# Autodesk Inventor assembly: ASY MSC 900.6 base frame
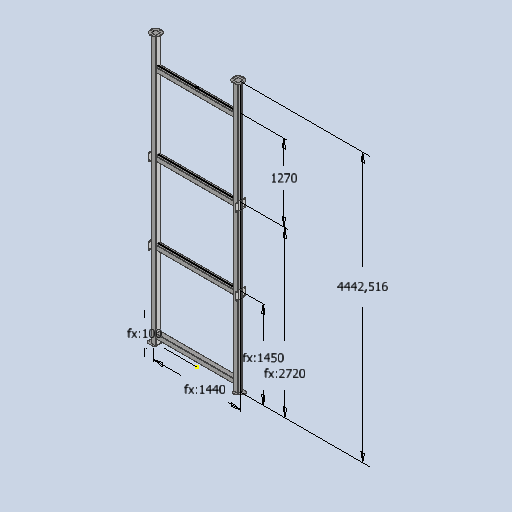
[picture p0: Inventor's stored thumbnail of the model, 512x512]
Saved by Autodesk Inventor 2025 (Build 290162010, 162A)
## iProperties
_SolveAssemblyDoc: Frame Generator Solve Assembly
_Version: 25.0.0
Created: 2024-06-30
Part Number: ASY MSC 900.6 base frame
Document SubType Name: Assembly
Designer: pokla
Stock Number: ASY МОО 900.6 базовая рама
Author: pokla
## Documents named in this file (6)
- C:\Users\DELL\YandexDisk-badmisterfox\домашниий пк\Inventor\Manturovo\Manturovo_Se-clar\Pillars\ASY MSC 900.6 base frame.iam
- C:\Users\DELL\YandexDisk-badmisterfox\домашниий пк\Inventor\Manturovo\Manturovo_Se-clar\Pillars\MSC DIM 009.6 base frame sketch.ipt
- C:\Users\DELL\YandexDisk-badmisterfox\домашниий пк\Inventor\Manturovo\Manturovo_Se-clar\Pillars\ASY MSC 900.6.1 base frame.iam
- C:\Users\DELL\YandexDisk-badmisterfox\домашниий пк\Inventor\Manturovo\Manturovo_Se-clar\MSC 902 flange frame heel.ipt
- C:\Users\DELL\YandexDisk-badmisterfox\домашниий пк\Inventor\Manturovo\Manturovo_Se-clar\MSC 906 flange frame.ipt
- C:\Users\DELL\YandexDisk-badmisterfox\домашниий пк\Inventor\Manturovo\Manturovo_Se-clar\MSC 908 transverse pillar plate.ipt
## Components (10 placed, 5 different names)
1. MSC DIM 009.6 base frame sketch:1
2. ASY MSC 900.6.1 base frame:1 [sub-assembly] — Rigid:3, Rigid:4, Rigid:5, Rigid:6, Rigid:7, Rigid:8, Rigid:9, Rigid:10
3. MSC 902 flange frame heel:1 — Rigid:5
4. MSC 902 flange frame heel:2 — Rigid:6
5. MSC 906 flange frame:1 — Rigid:3
6. MSC 906 flange frame:2 — Rigid:4
7. MSC 908 transverse pillar plate:1 — Rigid:7
8. MSC 908 transverse pillar plate:2 — Rigid:8
9. MSC 908 transverse pillar plate:3 — Rigid:9
10. MSC 908 transverse pillar plate:4 — Rigid:10
## Relationships (8: WeldJoint 8)
- Rigid:3 [WeldJoint]: ASY MSC 900.6.1 base frame:1 ↔ MSC 906 flange frame:1
- Rigid:4 [WeldJoint]: ASY MSC 900.6.1 base frame:1 ↔ MSC 906 flange frame:2
- Rigid:5 [WeldJoint]: ASY MSC 900.6.1 base frame:1 ↔ MSC 902 flange frame heel:1
- Rigid:6 [WeldJoint]: ASY MSC 900.6.1 base frame:1 ↔ MSC 902 flange frame heel:2
- Rigid:7 [WeldJoint] (80 mm): ASY MSC 900.6.1 base frame:1 ↔ MSC 908 transverse pillar plate:1
- Rigid:8 [WeldJoint] (80 mm): ASY MSC 900.6.1 base frame:1 ↔ MSC 908 transverse pillar plate:2
- Rigid:9 [WeldJoint] (80 mm): ASY MSC 900.6.1 base frame:1 ↔ MSC 908 transverse pillar plate:3
- Rigid:10 [WeldJoint] (80 mm): ASY MSC 900.6.1 base frame:1 ↔ MSC 908 transverse pillar plate:4
